# Autodesk Inventor assembly: MotorWheel
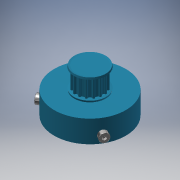
[picture p0: Inventor's stored thumbnail of the model, 180x180]
Saved by Autodesk Inventor 2018.3 (Build 223284000, 284)
## iProperties
Created: 2018-08-12
Part Number: MotorWheel
Material: Generisch
Document SubType Name: Assembly
Designer: JochenAlt
Author: JochenAlt
## Documents named in this file (6)
- D:\Projects\FlowerPot\CAD\Beltdrive\MotorWheel.iam
- D:\Projects\FlowerPot\CAD\Beltdrive\BeltDriveConstruction\Konstruktions-Assistent\Synchrone Riemenscheibe11.ipt
- D:\Projects\FlowerPot\CAD\Mounting Hub.ipt
- C:\Users\JochenAlt\Documents\Inventor\Content Center Files\R2018\de-DE\AS 1427(02)\AS 1427 - M3 x 6(2).ipt
- C:\Users\JochenAlt\Documents\Inventor\Content Center Files\R2018\de-DE\AS 1112 (4)\AS 1112 - M2(2).ipt
- C:\Users\JochenAlt\Documents\Inventor\Content Center Files\R2018\de-DE\DIN 912\DIN 912 - M2 x 0,4 x 3 x 2.ipt
## Components (13 placed, 5 different names)
1. Synchrone Riemenscheibe1:1 — Passend:4, Passend:5, Passend:6, Passend:7, Passend:8, Passend:9, Einfügen:8
2. Synchrone Riemenscheibe1:2 — Passend:1, Passend:2, Passend:3, Einfügen:1, Einfügen:2, Einfügen:3, Einfügen:4, Einfügen:5, Einfügen:6, Einfügen:7, Passend:4, Passend:5
3. Mounting Hub:1 — Passend:1, Passend:2, Passend:3
4. AS 1427 - Metrisch M3 x 6:1 — Einfügen:1
5. AS 1427 - Metrisch M3 x 6:2 — Einfügen:2
6. AS 1427 - Metrisch M3 x 6:3 — Einfügen:3
7. AS 1427 - Metrisch M3 x 6:4 — Einfügen:4
8. AS 1112 (4) - Metrisch M2:1 — Einfügen:5
9. AS 1112 (4) - Metrisch M2:2 — Einfügen:6
10. AS 1112 (4) - Metrisch M2:3 — Einfügen:7
11. DIN 912 - ersetzt durch DIN EN ISO 4762 M2 x 3:1 — Passend:6, Passend:7
12. DIN 912 - ersetzt durch DIN EN ISO 4762 M2 x 3:2 — Passend:8, Passend:9
13. DIN 912 - ersetzt durch DIN EN ISO 4762 M2 x 3:3 — Einfügen:8
## Relationships (17: Mate 9, Insert 8)
- Passend:1 [Mate]: Synchrone Riemenscheibe1:2 ↔ Mounting Hub:1
- Passend:2 [Mate]: Synchrone Riemenscheibe1:2 ↔ Mounting Hub:1
- Passend:3 [Mate]: Synchrone Riemenscheibe1:2 ↔ Mounting Hub:1
- Einfügen:1 [Insert]: Synchrone Riemenscheibe1:2 ↔ AS 1427 - Metrisch M3 x 6:1
- Einfügen:2 [Insert]: Synchrone Riemenscheibe1:2 ↔ AS 1427 - Metrisch M3 x 6:2
- Einfügen:3 [Insert]: Synchrone Riemenscheibe1:2 ↔ AS 1427 - Metrisch M3 x 6:3
- Einfügen:4 [Insert]: Synchrone Riemenscheibe1:2 ↔ AS 1427 - Metrisch M3 x 6:4
- Einfügen:5 [Insert]: Synchrone Riemenscheibe1:2 ↔ AS 1112 (4) - Metrisch M2:1
- Einfügen:6 [Insert]: Synchrone Riemenscheibe1:2 ↔ AS 1112 (4) - Metrisch M2:2
- Einfügen:7 [Insert]: Synchrone Riemenscheibe1:2 ↔ AS 1112 (4) - Metrisch M2:3
- Passend:4 [Mate]: Synchrone Riemenscheibe1:1 ↔ Synchrone Riemenscheibe1:2
- Passend:5 [Mate]: Synchrone Riemenscheibe1:1 ↔ Synchrone Riemenscheibe1:2
- Passend:6 [Mate]: Synchrone Riemenscheibe1:1 ↔ DIN 912 - ersetzt durch DIN EN ISO 4762 M2 x 3:1
- Passend:7 [Mate]: Synchrone Riemenscheibe1:1 ↔ DIN 912 - ersetzt durch DIN EN ISO 4762 M2 x 3:1
- Passend:8 [Mate]: Synchrone Riemenscheibe1:1 ↔ DIN 912 - ersetzt durch DIN EN ISO 4762 M2 x 3:2
- Passend:9 [Mate]: Synchrone Riemenscheibe1:1 ↔ DIN 912 - ersetzt durch DIN EN ISO 4762 M2 x 3:2
- Einfügen:8 [Insert]: Synchrone Riemenscheibe1:1 ↔ DIN 912 - ersetzt durch DIN EN ISO 4762 M2 x 3:3
